# Autodesk Inventor assembly: LightBracketAssembly
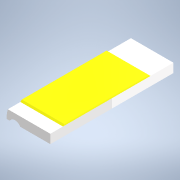
[picture p0: Inventor's stored thumbnail of the model, 180x180]
Saved by Autodesk Inventor 2021.2 (Build 252289000, 289)
## iProperties
Created: 2021-02-05
Part Number: LightBracketAssembly
Document SubType Name: Assembly
Designer: robst
Author: robst
## Documents named in this file (4)
- C:\git\CAD-Development\robSteele\HouseProjects\TrailerProjects\LightBracketAssembly.iam
- C:\git\CAD-Development\robSteele\HouseProjects\TrailerProjects\ketchenLightBracketV02-leftSide.ipt
- C:\git\CAD-Development\robSteele\HouseProjects\TrailerProjects\ketchenLightBracketV02-rightSide.ipt
- C:\git\CAD-Development\robSteele\HouseProjects\TrailerProjects\topForKetchenLight.ipt
## Components (3 placed, 3 different names)
1. ketchenLightBracketV02-leftSide:1 — Flush:1, Flush:2, Mate:1, Flush:3, Mate:2
2. ketchenLightBracketV02-rightSide:1 — Flush:1, Flush:2, Mate:2
3. topForKetchenLight:1 — Mate:1, Flush:3
## Relationships (5: Flush 3, Mate 2)
- Flush:1: ketchenLightBracketV02-leftSide:1 ↔ ketchenLightBracketV02-rightSide:1
- Flush:2: ketchenLightBracketV02-leftSide:1 ↔ ketchenLightBracketV02-rightSide:1
- Mate:1: ketchenLightBracketV02-leftSide:1 ↔ topForKetchenLight:1
- Flush:3: ketchenLightBracketV02-leftSide:1 ↔ topForKetchenLight:1
- Mate:2: ketchenLightBracketV02-leftSide:1 ↔ ketchenLightBracketV02-rightSide:1
